# Autodesk Inventor assembly: static_camera_slot
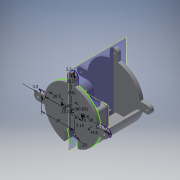
[picture p0: Inventor's stored thumbnail of the model, 180x180]
Saved by Autodesk Inventor 2019 (Build 230136000, 136)
## iProperties
Created: 2019-08-02
Part Number: static_camera_slot
Document SubType Name: Assembly
Designer: leode
Author: leode
## Documents named in this file (3)
- C:\Users\FTI\Documents\Digital Race\rplidar-a2m4-r1.stl\static_camera_slot.iam
- C:\Users\FTI\Documents\Digital Race\rplidar-a2m4-r1.stl\Astra_slot.ipt
- C:\Users\FTI\Documents\Digital Race\Camera_holder\Astra_perfect_top.ipt
## Components (2 placed, 2 different names)
1. Astra_slot:1 — Mate:1, Tangent:1, Flush:1
2. Astra_perfect_top:1 — Mate:1, Tangent:1, Flush:1
## Relationships (3: Mate 1, Tangent 1, Flush 1)
- Mate:1 (-3 mm): Astra_slot:1 ↔ Astra_perfect_top:1
- Tangent:1 (-20 mm): Astra_slot:1 ↔ Astra_perfect_top:1
- Flush:1: Astra_slot:1 ↔ Astra_perfect_top:1
